# Autodesk Inventor assembly: FY 15 TF
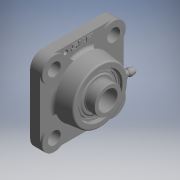
[picture p0: Inventor's stored thumbnail of the model, 180x180]
Saved by Autodesk Inventor 2017.3 (Build 213256000, 256)
## iProperties
Category: PARTsolutions
Company: SKF
Part Number: FY 15 TF
Catalog Web Link: www.cadenas.de
Description: AYF_001HC_HH_HY-Y-bearing square flanged units
Vendor: SKF
Document SubType Name: Assembly
Designer: partserver
Manufacturer: SKF
Mass: 370 g
Surface Area: 342.54 cm^2
Volume: 53.3408 cm^3
Density: 6.93652 g/cm^3
Title: FY 15 TF
Author: Cadenas PARTsolutions
Comments: Y-bearing square flanged units
PSOL_IDENT_0: {$CADENAS_DATA\23d-libs\skf\bearings_units_and_housings\bearing_units\ball_bearing_units\y-units\ayf
PSOL_IDENT_1: _001hc_hh_hy.prj},187 {VTYP=3D},{STYP=ASSTAB},{NB=FY 15 TF},{LINA=FY 15 TF},{NN=AYF_001HC_HH_HY},{DA
PSOL_IDENT_2: TE=20.08.2020 12:22:38},{GEOMDATE=20.08.2020 12:22:32},{VERSION=},{LINEID=58220},{WBVAR=COVER},{WBNU
PSOL_IDENT_3: MERIC=}  {NB=FY 15 TF},{LINA=FY 15 TF},{KT=DUMMY},{DESIGNATION=FY 15 TF},{HOUSING=FY 503 M},{BEARING=
PSOL_IDENT_4: YAR 203/15-2F},{COVER=},{DD=15},{DDX=},{DDALG=15.000},{DD1=24.200},{DD2=MIN},{DD3=},{AALG=26.000},{A=
PSOL_IDENT_5: 26},{AX=},{AXX=},{A1ALG=11.000},{A1=11},{A1X=},{A1XX=},{A3ALG=3.200},{A3=3.2},{A3X=},{A5ALG=0.000},{
PSOL_IDENT_6: A5=},{A5X=},{A5XX=},{B=27.400},{B1=MIN},{B1X=},{B4ALG=4.000},{B4=4},{B4X=},{DAAALG=55.600},{DAA=55.6
PSOL_IDENT_7: },{DAAX=},{DB=MIN},{DB1=50.000},{DB1X=},{DB2=53.000},{DB2X=},{HA=},{J=54.000},{JX=},{JXX=},{L=76.000
PSOL_IDENT_8: },{LX=},{LXX=},{N=11.500},{NX=},{NXX=},{SS1=15.900},{SS1X=},{T=32.900},{TX=},{DN=6.500},{SWN=7},{GN=
PSOL_IDENT_9: 1/4-28 SAE-LT},{RG=1/4-28 UNF},{RGX=},{R1=19},{R1X=},{J6=66},{J7=14.500},{N4=4},{D=40.000},{C=12.000
PSOL_IDENT_10: },{R12=0.300},{DW=6.747},{B3=MIN},{PITCH=28.500},{LOAD1=9.560},{LOAD2=4.750},{LOAD3=0.200},{SPEED1=9
PSOL_IDENT_11: 500},{II=1},{Z=8},{MASS=0.370},{MASSX=},{G2=M6x0.75},{HKSGS=3},{RTTGS=4},{ALPHA=},{GALG=10.000},{G=1
PSOL_IDENT_12: 0},{GX=},{GXX=},{GINALG=0.375},{GIN=0.375000002475},{GINX=},{GINXX=},{EC=},{BS=},{SLEEVE=},{POPULAR=
PSOL_IDENT_13: },{D1=MIN},{K=},{CC1=},{BRGTYP=BBY_006},{COVERALG=  '', 'No end cover' },{SUPPRESSED=unsuppressed},{
PSOL_IDENT_14: TC=FY 15 TF},{PPATH=y-bearing_square_flanged_units_parts/ayf_001hc_hh_hy_asmtpl.prj}
NB: FY 15 TF
NN: AYF_001HC_HH_HY
NT: Y-bearing square flanged units
NBSYN: $TC.
LINA: FY 15 TF
CATALOG: SKF
DESIGNATION: FY 15 TF
HOUSING: FY 503 M
BEARING: YAR 203/15-2F
COVER: No end cover
DDALG: 15
J: 54
L: 76
T: 32.9
LOAD1: 9.56
LOAD2: 4.75
SPEED1: 9500
SUPPLIER: SKF
ARTICLENO: FY 15 TF
BOMINFO: FY 15 TF
CREATOR: CADENAS GmbH
## Documents named in this file (6)
- e:\temp\worker_99\temp\exporttempdir_4692_6_LMKB5\format_0\FY 15 TF.iam
- e:\temp\worker_99\temp\exporttempdir_4692_6_LMKB5\format_0\FY 17 TF0_375000002475-dummy.ipt
- e:\temp\worker_99\temp\exporttempdir_4692_6_LMKB5\format_0\FY 503 M-housing.ipt
- e:\temp\worker_99\temp\exporttempdir_4692_6_LMKB5\format_0\1_4-28 SAE-LT.ipt
- e:\temp\worker_99\temp\exporttempdir_4692_6_LMKB5\format_0\YAR 203-2F-24_210300220312 -bearing.ipt
- e:\temp\worker_99\temp\exporttempdir_4692_6_LMKB5\format_0\17-40-27_4-12-ybrg1-43-6_747-28_5.ipt
## Components (12 placed, 5 different names)
1. FY 17 TF0_375000002475-dummy:1 — brg_XY@1 <-> housing_XY@2, brg_Z@1 <-> housing_Z@2, brg_YZ@1 <-> housing_YZ@2
2. FY 503 M-housing:1 — brg_XY@1 <-> housing_XY@2, brg_Z@1 <-> housing_Z@2, brg_YZ@1 <-> housing_YZ@2, gn_XY@2 <-> gn_XY@3, gn_Z@2 <-> gn_Z@3, gn_YZ@2 <-> gn_YZ@3, housing_XY@2 <-> brg3_XY@4, housing_Z@2 <-> brg3_Z@4, housing_YZ@2 <-> brg3_YZ@4
3. 1_4-28 SAE-LT:1 — gn_XY@2 <-> gn_XY@3, gn_Z@2 <-> gn_Z@3, gn_YZ@2 <-> gn_YZ@3
4. YAR 203-2F-24_210300220312 -bearing:1 — housing_XY@2 <-> brg3_XY@4, housing_Z@2 <-> brg3_Z@4, housing_YZ@2 <-> brg3_YZ@4, ball_1_XY@4 <-> ball_XY@5, ball_1_Z@4 <-> ball_Z@5, ball_1_YZ@4 <-> ball_YZ@5, ball_2_XY@4 <-> ball_XY@6, ball_2_Z@4 <-> ball_Z@6, ball_2_YZ@4 <-> ball_YZ@6, ball_3_XY@4 <-> ball_XY@7, ball_3_Z@4 <-> ball_Z@7, ball_3_YZ@4 <-> ball_YZ@7, ball_4_XY@4 <-> ball_XY@8, ball_4_Z@4 <-> ball_Z@8, ball_4_YZ@4 <-> ball_YZ@8, ball_5_XY@4 <-> ball_XY@9, ball_5_Z@4 <-> ball_Z@9, ball_5_YZ@4 <-> ball_YZ@9, ball_6_XY@4 <-> ball_XY@10, ball_6_Z@4 <-> ball_Z@10, ball_6_YZ@4 <-> ball_YZ@10, ball_7_XY@4 <-> ball_XY@11, ball_7_Z@4 <-> ball_Z@11, ball_7_YZ@4 <-> ball_YZ@11, ball_8_XY@4 <-> ball_XY@12, ball_8_Z@4 <-> ball_Z@12, ball_8_YZ@4 <-> ball_YZ@12
5. 17-40-27_4-12-ybrg1-43-6_747-28_5:1 — ball_1_XY@4 <-> ball_XY@5, ball_1_Z@4 <-> ball_Z@5, ball_1_YZ@4 <-> ball_YZ@5
6. 17-40-27_4-12-ybrg1-43-6_747-28_5:2 — ball_2_XY@4 <-> ball_XY@6, ball_2_Z@4 <-> ball_Z@6, ball_2_YZ@4 <-> ball_YZ@6
7. 17-40-27_4-12-ybrg1-43-6_747-28_5:3 — ball_3_XY@4 <-> ball_XY@7, ball_3_Z@4 <-> ball_Z@7, ball_3_YZ@4 <-> ball_YZ@7
8. 17-40-27_4-12-ybrg1-43-6_747-28_5:4 — ball_4_XY@4 <-> ball_XY@8, ball_4_Z@4 <-> ball_Z@8, ball_4_YZ@4 <-> ball_YZ@8
9. 17-40-27_4-12-ybrg1-43-6_747-28_5:5 — ball_5_XY@4 <-> ball_XY@9, ball_5_Z@4 <-> ball_Z@9, ball_5_YZ@4 <-> ball_YZ@9
10. 17-40-27_4-12-ybrg1-43-6_747-28_5:6 — ball_6_XY@4 <-> ball_XY@10, ball_6_Z@4 <-> ball_Z@10, ball_6_YZ@4 <-> ball_YZ@10
11. 17-40-27_4-12-ybrg1-43-6_747-28_5:7 — ball_7_XY@4 <-> ball_XY@11, ball_7_Z@4 <-> ball_Z@11, ball_7_YZ@4 <-> ball_YZ@11
12. 17-40-27_4-12-ybrg1-43-6_747-28_5:8 — ball_8_XY@4 <-> ball_XY@12, ball_8_Z@4 <-> ball_Z@12, ball_8_YZ@4 <-> ball_YZ@12
## Relationships (33: Mate 21, Angle 11, Flush 1)
- brg_XY@1 <-> housing_XY@2 [Mate]: FY 17 TF0_375000002475-dummy:1 ↔ FY 503 M-housing:1
- brg_Z@1 <-> housing_Z@2 [Mate]: FY 17 TF0_375000002475-dummy:1 ↔ FY 503 M-housing:1
- brg_YZ@1 <-> housing_YZ@2 [Angle] (180 deg): FY 17 TF0_375000002475-dummy:1 ↔ FY 503 M-housing:1
- gn_XY@2 <-> gn_XY@3 [Mate]: FY 503 M-housing:1 ↔ 1_4-28 SAE-LT:1
- gn_Z@2 <-> gn_Z@3 [Mate]: FY 503 M-housing:1 ↔ 1_4-28 SAE-LT:1
- gn_YZ@2 <-> gn_YZ@3 [Angle] (0 deg): FY 503 M-housing:1 ↔ 1_4-28 SAE-LT:1
- housing_XY@2 <-> brg3_XY@4 [Flush] (32.9 mm): FY 503 M-housing:1 ↔ YAR 203-2F-24_210300220312 -bearing:1
- housing_Z@2 <-> brg3_Z@4 [Mate]: FY 503 M-housing:1 ↔ YAR 203-2F-24_210300220312 -bearing:1
- housing_YZ@2 <-> brg3_YZ@4 [Angle] (0 deg): FY 503 M-housing:1 ↔ YAR 203-2F-24_210300220312 -bearing:1
- ball_1_XY@4 <-> ball_XY@5 [Mate]: YAR 203-2F-24_210300220312 -bearing:1 ↔ 17-40-27_4-12-ybrg1-43-6_747-28_5:1
- ball_1_Z@4 <-> ball_Z@5 [Mate]: YAR 203-2F-24_210300220312 -bearing:1 ↔ 17-40-27_4-12-ybrg1-43-6_747-28_5:1
- ball_1_YZ@4 <-> ball_YZ@5 [Angle] (0 deg): YAR 203-2F-24_210300220312 -bearing:1 ↔ 17-40-27_4-12-ybrg1-43-6_747-28_5:1
- ball_2_XY@4 <-> ball_XY@6 [Mate]: YAR 203-2F-24_210300220312 -bearing:1 ↔ 17-40-27_4-12-ybrg1-43-6_747-28_5:2
- ball_2_Z@4 <-> ball_Z@6 [Mate]: YAR 203-2F-24_210300220312 -bearing:1 ↔ 17-40-27_4-12-ybrg1-43-6_747-28_5:2
- ball_2_YZ@4 <-> ball_YZ@6 [Angle] (0 deg): YAR 203-2F-24_210300220312 -bearing:1 ↔ 17-40-27_4-12-ybrg1-43-6_747-28_5:2
- ball_3_XY@4 <-> ball_XY@7 [Mate]: YAR 203-2F-24_210300220312 -bearing:1 ↔ 17-40-27_4-12-ybrg1-43-6_747-28_5:3
- ball_3_Z@4 <-> ball_Z@7 [Mate]: YAR 203-2F-24_210300220312 -bearing:1 ↔ 17-40-27_4-12-ybrg1-43-6_747-28_5:3
- ball_3_YZ@4 <-> ball_YZ@7 [Angle] (0 deg): YAR 203-2F-24_210300220312 -bearing:1 ↔ 17-40-27_4-12-ybrg1-43-6_747-28_5:3
- ball_4_XY@4 <-> ball_XY@8 [Mate]: YAR 203-2F-24_210300220312 -bearing:1 ↔ 17-40-27_4-12-ybrg1-43-6_747-28_5:4
- ball_4_Z@4 <-> ball_Z@8 [Mate]: YAR 203-2F-24_210300220312 -bearing:1 ↔ 17-40-27_4-12-ybrg1-43-6_747-28_5:4
- ball_4_YZ@4 <-> ball_YZ@8 [Angle] (0 deg): YAR 203-2F-24_210300220312 -bearing:1 ↔ 17-40-27_4-12-ybrg1-43-6_747-28_5:4
- ball_5_XY@4 <-> ball_XY@9 [Mate]: YAR 203-2F-24_210300220312 -bearing:1 ↔ 17-40-27_4-12-ybrg1-43-6_747-28_5:5
- ball_5_Z@4 <-> ball_Z@9 [Mate]: YAR 203-2F-24_210300220312 -bearing:1 ↔ 17-40-27_4-12-ybrg1-43-6_747-28_5:5
- ball_5_YZ@4 <-> ball_YZ@9 [Angle] (0 deg): YAR 203-2F-24_210300220312 -bearing:1 ↔ 17-40-27_4-12-ybrg1-43-6_747-28_5:5
- ball_6_XY@4 <-> ball_XY@10 [Mate]: YAR 203-2F-24_210300220312 -bearing:1 ↔ 17-40-27_4-12-ybrg1-43-6_747-28_5:6
- ball_6_Z@4 <-> ball_Z@10 [Mate]: YAR 203-2F-24_210300220312 -bearing:1 ↔ 17-40-27_4-12-ybrg1-43-6_747-28_5:6
- ball_6_YZ@4 <-> ball_YZ@10 [Angle] (0 deg): YAR 203-2F-24_210300220312 -bearing:1 ↔ 17-40-27_4-12-ybrg1-43-6_747-28_5:6
- ball_7_XY@4 <-> ball_XY@11 [Mate]: YAR 203-2F-24_210300220312 -bearing:1 ↔ 17-40-27_4-12-ybrg1-43-6_747-28_5:7
- ball_7_Z@4 <-> ball_Z@11 [Mate]: YAR 203-2F-24_210300220312 -bearing:1 ↔ 17-40-27_4-12-ybrg1-43-6_747-28_5:7
- ball_7_YZ@4 <-> ball_YZ@11 [Angle] (0 deg): YAR 203-2F-24_210300220312 -bearing:1 ↔ 17-40-27_4-12-ybrg1-43-6_747-28_5:7
- ball_8_XY@4 <-> ball_XY@12 [Mate]: YAR 203-2F-24_210300220312 -bearing:1 ↔ 17-40-27_4-12-ybrg1-43-6_747-28_5:8
- ball_8_Z@4 <-> ball_Z@12 [Mate]: YAR 203-2F-24_210300220312 -bearing:1 ↔ 17-40-27_4-12-ybrg1-43-6_747-28_5:8
- ball_8_YZ@4 <-> ball_YZ@12 [Angle] (0 deg): YAR 203-2F-24_210300220312 -bearing:1 ↔ 17-40-27_4-12-ybrg1-43-6_747-28_5:8
